# Autodesk Inventor assembly: C-TFK10
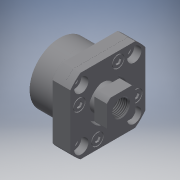
[picture p0: Inventor's stored thumbnail of the model, 180x180]
Saved by Autodesk Inventor 2019 (Build 230136000, 136)
## iProperties
Category: PARTsolutions
Company: MISUMI
Created: 2023-03-01
Part Number: C-TFK10
Catalog Web Link: www.cadenas.de
Description: C-TFK-Economy Support Units Fixed Side Round
Vendor: MISUMI
Document SubType Name: Assembly
Designer: psAdmin
Manufacturer: MISUMI
Mass: 29.2483 g
Surface Area: 108.462 cm^2
Volume: 29.2483 cm^3
Density: 1 g/cm^3
Title: C-TFK10
Author: Cadenas PARTsolutions
Comments: Economy Support Units Fixed Side Round
PSOL_IDENT_0: {$CADENAS_DATA/23d-libs/misumi/metric/09_ball_screws/c_tfk_asmtab.prj},171 {VTYP=3D},{STYP=ASSTAB},{
PSOL_IDENT_1: NB=C-TFK10},{LINA=C-TFK10},{NN=C-TFK},{DATE=14.09.2022 01:45:34},{GEOMDATE=16.11.2021 00:43:58},{VER
PSOL_IDENT_2: SION=},{LINEID=100},{WBVAR=SET},{WBNUMERIC=}  {NB=C-TFK10},{LINA=C-TFK10},{KT=DUMMY},{PN=C-TFK10},{T
PSOL_IDENT_3: YPE=C-TFK},{NO=10},{SET=},{DD=10},{L=27},{H=10},{F=17},{E=29.5},{D=34},{A=52},{PCD=42},{B=42},{L1=7.
PSOL_IDENT_4: 5},{T1=5.0},{DD1=4.5},{DD2=8.0},{LL=4.0},{M=M10x1.0},{T=16},{SID=14.0},{Z1=22},{Z2=14.5},{Z3=6.0},{Z
PSOL_IDENT_5: 4=3.0},{Z5=21},{X1=7},{X2=6.2},{X3=3.00},{X4=34},{CP=10},{Y1=0},{Y2=0.0},{Y3=0.0},{Y4=0},{B1=2.3},{B
PSOL_IDENT_6: 2=4.55},{NO2=10},{PPATH=c_tfk/c_tfk_asmtpl.prj},{SETALG= '', 'w/o SET', '-SET', 'with SET' },{ACD=14
PSOL_IDENT_7: .5},{ACV=10},{ACL=5.5},{ACNM=M10x1.0},{ACNB=8.0},{ACNMM=M3},{ACNDD=15},{ACND=20.0},{ACNF=16}
NB: C-TFK10
NN: C-TFK
NT: Economy Support Units Fixed Side Round
NBSYN: $PN.
LINA: C-TFK10
CATALOG: Misumi
PN: C-TFK10
NO: 10
SET: w/o SET
DD: 10
L: 27
H: 10
F: 17
E: 29.5
D: 34
A: 52
PCD: 42
B: 42
L1: 7.5
T1: 5
DD1: 4.5
DD2: 8
LL: 4
M: M10x1.0
T: 16
ACD: 14.5
ACV: 10
ACL: 5.5
ACNM: M10x1.0
ACNB: 8
ACNMM: M3
ACNDD: 15
ACND: 20
ACNF: 16
SUPPLIER: MISUMI
ARTICLENO: C-TFK10
BOMINFO: C-TFK10
CREATOR: CADENAS GmbH
## Documents named in this file (4)
- e:\temp\worker_COMMON_3\temp\tmp_4476_64_R9Msm\format_0\C-TFK10.iam
- e:\temp\worker_COMMON_3\temp\tmp_4476_64_R9Msm\format_0\C-TFK10_b.ipt
- e:\temp\worker_COMMON_3\temp\tmp_4476_64_R9Msm\format_0\C-TFK10_c.ipt
- e:\temp\worker_COMMON_3\temp\tmp_4476_64_R9Msm\format_0\C-TFK10_n.ipt
## Components (4 placed, 3 different names)
1. C-TFK10_b:1 — to_collar_XY@1 <-> to_base_XY@2, to_collar_Z@1 <-> to_base_Z@2, to_collar_YZ@1 <-> to_base_YZ@2, to_collar_2_XY@1 <-> to_base_XY@4, to_collar_2_Z@1 <-> to_base_Z@4, to_collar_2_YZ@1 <-> to_base_YZ@4
2. C-TFK10_c:1 — to_collar_XY@1 <-> to_base_XY@2, to_collar_Z@1 <-> to_base_Z@2, to_collar_YZ@1 <-> to_base_YZ@2, to_nut_XY@2 <-> to_collar_XY@3, to_nut_Z@2 <-> to_collar_Z@3, to_nut_YZ@2 <-> to_collar_YZ@3
3. C-TFK10_n:1 — to_nut_XY@2 <-> to_collar_XY@3, to_nut_Z@2 <-> to_collar_Z@3, to_nut_YZ@2 <-> to_collar_YZ@3
4. C-TFK10_c:2 — to_collar_2_XY@1 <-> to_base_XY@4, to_collar_2_Z@1 <-> to_base_Z@4, to_collar_2_YZ@1 <-> to_base_YZ@4
## Relationships (9: Mate 6, Angle 3)
- to_collar_XY@1 <-> to_base_XY@2 [Mate]: C-TFK10_b:1 ↔ C-TFK10_c:1
- to_collar_Z@1 <-> to_base_Z@2 [Mate]: C-TFK10_b:1 ↔ C-TFK10_c:1
- to_collar_YZ@1 <-> to_base_YZ@2 [Angle] (0 deg): C-TFK10_b:1 ↔ C-TFK10_c:1
- to_nut_XY@2 <-> to_collar_XY@3 [Mate]: C-TFK10_c:1 ↔ C-TFK10_n:1
- to_nut_Z@2 <-> to_collar_Z@3 [Mate]: C-TFK10_c:1 ↔ C-TFK10_n:1
- to_nut_YZ@2 <-> to_collar_YZ@3 [Angle] (45 deg): C-TFK10_c:1 ↔ C-TFK10_n:1
- to_collar_2_XY@1 <-> to_base_XY@4 [Mate]: C-TFK10_b:1 ↔ C-TFK10_c:2
- to_collar_2_Z@1 <-> to_base_Z@4 [Mate]: C-TFK10_b:1 ↔ C-TFK10_c:2
- to_collar_2_YZ@1 <-> to_base_YZ@4 [Angle] (0 deg): C-TFK10_b:1 ↔ C-TFK10_c:2
